# Autodesk Inventor assembly: FullSailCapstan-ver2-1111-2021
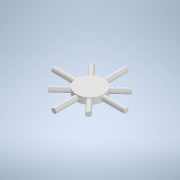
[picture p0: Inventor's stored thumbnail of the model, 180x180]
Saved by Autodesk Inventor 2021 (Build 250183000, 183)
## iProperties
Created: 2021-03-03
Part Number: FullSailCapstan-ver2-1111-2021
Document SubType Name: Assembly
Designer: CMurray
Author: CMurray
## Documents named in this file (3)
- F:\PHRC CADD 2021\2021 Game Design Challenge\Crow's Nest\Parts\Capstan\FullSailCapstan-ver2-1111-2021.iam
- F:\PHRC CADD 2021\2021 Game Design Challenge\Crow's Nest\Parts\Capstan\CapMid-ver1-1111-2021.ipt
- F:\PHRC CADD 2021\2021 Game Design Challenge\Crow's Nest\Parts\Capstan\CapMid-ver2-1111-2021.ipt
## Components (2 placed, 2 different names)
1. CapMid-ver1-1111-2021:1 — Rotational:1
2. CapMid-ver2-1111-2021:1 — Rotational:1
## Relationships (1: RevoluteJoint 1)
- Rotational:1 [RevoluteJoint]: CapMid-ver1-1111-2021:1 ↔ CapMid-ver2-1111-2021:1
